# Autodesk Inventor assembly: main_idea
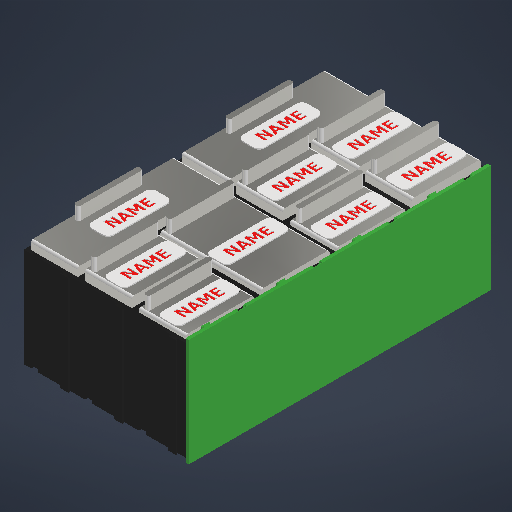
[picture p0: Inventor's stored thumbnail of the model, 512x512]
Saved by Autodesk Inventor 2027 (Build 310192060, 192F)
## iProperties
Created: 2026-06-08
Part Number: main_idea
Document SubType Name: Assembly
Designer: User
Author: User
## Documents named in this file (8)
- C:\Users\Duszy\Desktop\Modular_shelf\main_idea.iam
- C:\Users\Duszy\Desktop\Modular_shelf\Parts\box1x1.ipt
- C:\Users\Duszy\Desktop\Modular_shelf\Parts\box1x2.ipt
- C:\Users\Duszy\Desktop\Modular_shelf\Parts\box2x1.ipt
- C:\Users\Duszy\Desktop\Modular_shelf\Parts\shelf1x1.ipt
- C:\Users\Duszy\Desktop\Modular_shelf\Parts\shelf2x1.ipt
- C:\Users\Duszy\Desktop\Modular_shelf\Parts\shelf1x2.ipt
- C:\Users\Duszy\Desktop\Modular_shelf\Parts\Edge.ipt
## Components (22 placed, 7 different names)
1. box1x2:1 — Sztywne:1, Sztywne:2, Walcowe:2
2. shelf2x1:1 — Walcowe:2
3. box2x1:1 — Sztywne:3, Walcowe:4
4. shelf1x2:1 — Walcowe:4
5. box2x1:2
6. shelf1x2:2
7. shelf1x1:2 — Walcowe:3
8. box1x1:2 — Sztywne:2, Sztywne:3, Walcowe:3
9. shelf1x1:1 — Walcowe:1
10. box1x1:1 — Sztywne:1, Walcowe:1, Sztywne:5
11. shelf1x1:3
12. box1x1:3 — Sztywne:4
13. shelf1x1:4
14. box1x1:4
15. box1x1:5 — Sztywne:4
16. shelf1x1:5
17. box1x1:6
18. shelf1x1:6
19. Edge:1 — Sztywne:5
20. Edge:2
21. Edge:3
22. Edge:4
## Component patterns: (2 elements, first: box2x1:1 + shelf1x2:1), (2 elements, first: shelf1x1:2 + box1x1:2 + shelf1x1:1 + box1x1:1), (2 elements, first: box1x1:5 + shelf1x1:5), (4 elements, first: Edge:1)
## Relationships (10: WeldJoint 5, CylindricalJoint 5)
- Sztywne:1 [WeldJoint] (0.2 mm): box1x2:1 ↔ box1x1:1
- Sztywne:2 [WeldJoint] (0.2 mm): box1x2:1 ↔ box1x1:2
- Sztywne:3 [WeldJoint] (0.2 mm): box2x1:1 ↔ box1x1:2
- Walcowe:1 [CylindricalJoint]: shelf1x1:1 ↔ box1x1:1
- Walcowe:2 [CylindricalJoint]: box1x2:1 ↔ shelf2x1:1
- Walcowe:3 [CylindricalJoint]: shelf1x1:2 ↔ box1x1:2
- Walcowe:4 [CylindricalJoint]: box2x1:1 ↔ shelf1x2:1
- [CylindricalJoint]: box1x1:5 ↔ shelf1x1:5
- Sztywne:4 [WeldJoint] (0.2 mm): box1x1:3 ↔ box1x1:5
- Sztywne:5 [WeldJoint] (0.2 mm): box1x1:1 ↔ Edge:1
## Named parameters: d79_d57 = 180 deg, d80_d58 = 180 deg, d81_d59 = 180 deg, d82_d61 = 7.59745 mm, d83_d63 = 0 mm, d84_d64 = 0 mm
